# Autodesk Inventor assembly: Alliance Marker - Red
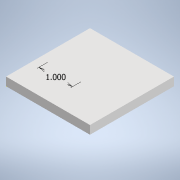
[picture p0: Inventor's stored thumbnail of the model, 180x180]
Saved by Autodesk Inventor 2020 (Build 240168000, 168)
## iProperties
Created: 2020-01-17
Part Number: Alliance Marker - Red
Document SubType Name: Assembly
Designer: maple
Author: maple
## Documents named in this file (3)
- C:\Users\maple\Documents\GitHub\3D-Models\Robotics\Alliance Marker - Red.iam
- C:\Users\maple\Documents\GitHub\3D-Models\Robotics\Alliance Marker - Red.ipt
- C:\Users\maple\Documents\GitHub\3D-Models\Robotics\Mount Male.ipt
## Components (2 placed, 2 different names)
1. Alliance Marker - Red:1 — Rigid:1
2. Mount Male:1 — Rigid:1
## Relationships (1: WeldJoint 1)
- Rigid:1 [WeldJoint] (1.5875 mm): Alliance Marker - Red:1 ↔ Mount Male:1
